# Autodesk Inventor assembly: MainAssembly
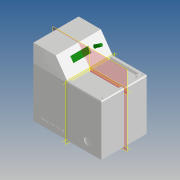
[picture p0: Inventor's stored thumbnail of the model, 180x180]
Saved by Autodesk Inventor 2020.4 (Build 244396000, 396)
## iProperties
Created: 2022-05-18
Part Number: MainAssembly
Document SubType Name: Assembly
Designer: Lukas
Author: Lukas
## Documents named in this file (5)
- D:\school\Inventor\projecten\Case\MainAssembly.iam
- D:\school\Inventor\projecten\Case\bigBoard.ipt
- D:\school\Inventor\projecten\Case\caseBottom.ipt
- D:\school\Inventor\projecten\Case\deksel.ipt
- D:\school\Inventor\projecten\Case\smallBoard.ipt
## Components (4 placed, 4 different names)
1. bigBoard:1 — Insert:1, Insert:2
2. caseBottom:1 — Insert:1, Insert:2, Mate:1, Mate:2, Mate:3
3. deksel:1 — Mate:1, Mate:2, Mate:3, Mate:4, Mate:5, Mate:6
4. smallBoard:1 — Mate:4, Mate:5, Mate:6
## Relationships (8: Mate 6, Insert 2)
- Insert:1: bigBoard:1 ↔ caseBottom:1
- Insert:2: bigBoard:1 ↔ caseBottom:1
- Mate:1: caseBottom:1 ↔ deksel:1
- Mate:2: caseBottom:1 ↔ deksel:1
- Mate:3: caseBottom:1 ↔ deksel:1
- Mate:4 (7 mm): deksel:1 ↔ smallBoard:1
- Mate:5: deksel:1 ↔ smallBoard:1
- Mate:6: deksel:1 ↔ smallBoard:1
